# Autodesk Inventor assembly: Silver
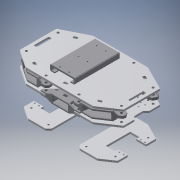
[picture p0: Inventor's stored thumbnail of the model, 180x180]
Saved by Autodesk Inventor 2016 (Build 200138000, 138)
## iProperties
Created: 2016-09-29
Part Number: Silver
Material: Générique
Document SubType Name: Assembly
Designer: LogOut
Author: LogOut
## Documents named in this file (10)
- C:\Travail\Objets\GitHub\Silver\Mechanic\Silver.iam
- C:\Travail\Objets\GitHub\Silver\Mechanic\Support_Roue.ipt
- C:\Travail\Objets\GitHub\Silver\Mechanic\Support_Moteur.ipt
- C:\Travail\Objets\GitHub\Silver\Mechanic\Support_GP2.C.ipt
- C:\Travail\Objets\GitHub\Silver\Mechanic\Support_Carte.ipt
- C:\Travail\Objets\GitHub\Silver\Mechanic\Support_GP2.Av.ipt
- C:\Travail\Objets\GitHub\Silver\Mechanic\Support_GP2.Av_MIR1.ipt
- C:\Travail\Objets\GitHub\Silver\Mechanic\Support_GP2.Ar.ipt
- C:\Travail\Objets\GitHub\Silver\Mechanic\Support_GP2.Ar_MIR.ipt
- C:\Travail\Objets\GitHub\Silver\Mechanic\Support_logique.ipt
## Components (11 placed, 9 different names)
1. Support_Roue:1 — Placage:2, Placage:13, Placage:14
2. Support_Roue:2 — Placage:1, Placage:11, Placage:12
3. Support_Moteur:1 — Placage:1, Placage:2, Placage:11, Placage:12, Placage:13, Placage:14, Placage:15, Affleurement:1, Affleurement:2, Placage:16, Placage:17, Placage:18, Placage:20, Placage:21, Placage:22
4. Support_Carte:1 — Placage:15, Affleurement:1, Affleurement:2, Placage:23, Placage:24, Placage:28, Placage:29, Placage:30, Placage:31, Placage:32, Placage:33, Placage:34, Affleurement:6, Placage:35, Affleurement:7
5. Support_GP2.C:1 — Placage:20, Placage:21, Placage:22
6. Support_GP2.C:2 — Placage:16, Placage:17, Placage:18
7. Support_GP2.Av:1 — Placage:23, Placage:24, Placage:28, Affleurement:3
8. Support_GP2.Av_MIR1:1 — Affleurement:3, Placage:29, Placage:30, Affleurement:4
9. Support_GP2.Ar:1 — Affleurement:4, Placage:31, Placage:32, Affleurement:5
10. Support_GP2.Ar_MIR:1 — Affleurement:5, Placage:33, Placage:34
11. Support_logique:1 — Affleurement:6, Placage:35, Affleurement:7
## Relationships (30: Mate 23, Flush 7)
- Placage:1 [Mate] (100 mm): Support_Roue:2 ↔ Support_Moteur:1
- Placage:2 [Mate] (100 mm): Support_Roue:1 ↔ Support_Moteur:1
- Placage:11 [Mate]: Support_Roue:2 ↔ Support_Moteur:1
- Placage:12 [Mate]: Support_Roue:2 ↔ Support_Moteur:1
- Placage:13 [Mate]: Support_Roue:1 ↔ Support_Moteur:1
- Placage:14 [Mate]: Support_Roue:1 ↔ Support_Moteur:1
- Placage:15 [Mate] (40 mm): Support_Moteur:1 ↔ Support_Carte:1
- Affleurement:1 [Flush]: Support_Moteur:1 ↔ Support_Carte:1
- Affleurement:2 [Flush]: Support_Moteur:1 ↔ Support_Carte:1
- Placage:16 [Mate]: Support_Moteur:1 ↔ Support_GP2.C:2
- Placage:17 [Mate]: Support_Moteur:1 ↔ Support_GP2.C:2
- Placage:18 [Mate]: Support_Moteur:1 ↔ Support_GP2.C:2
- Placage:20 [Mate]: Support_Moteur:1 ↔ Support_GP2.C:1
- Placage:21 [Mate]: Support_Moteur:1 ↔ Support_GP2.C:1
- Placage:22 [Mate]: Support_Moteur:1 ↔ Support_GP2.C:1
- Placage:23 [Mate]: Support_Carte:1 ↔ Support_GP2.Av:1
- Placage:24 [Mate]: Support_Carte:1 ↔ Support_GP2.Av:1
- Placage:28 [Mate] (4 mm): Support_Carte:1 ↔ Support_GP2.Av:1
- Affleurement:3 [Flush]: Support_GP2.Av:1 ↔ Support_GP2.Av_MIR1:1
- Placage:29 [Mate]: Support_Carte:1 ↔ Support_GP2.Av_MIR1:1
- Placage:30 [Mate]: Support_Carte:1 ↔ Support_GP2.Av_MIR1:1
- Affleurement:4 [Flush]: Support_GP2.Av_MIR1:1 ↔ Support_GP2.Ar:1
- Placage:31 [Mate]: Support_Carte:1 ↔ Support_GP2.Ar:1
- Placage:32 [Mate]: Support_Carte:1 ↔ Support_GP2.Ar:1
- Affleurement:5 [Flush]: Support_GP2.Ar:1 ↔ Support_GP2.Ar_MIR:1
- Placage:33 [Mate]: Support_Carte:1 ↔ Support_GP2.Ar_MIR:1
- Placage:34 [Mate]: Support_Carte:1 ↔ Support_GP2.Ar_MIR:1
- Affleurement:6 [Flush] (10 mm): Support_Carte:1 ↔ Support_logique:1
- Placage:35 [Mate] (20 mm): Support_Carte:1 ↔ Support_logique:1
- Affleurement:7 [Flush] (129 mm): Support_Carte:1 ↔ Support_logique:1
